# Autodesk Inventor assembly: chassis_assembly.ipt
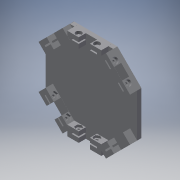
[picture p0: Inventor's stored thumbnail of the model, 180x180]
Saved by Autodesk Inventor 2018 (Build 220112000, 112)
## iProperties
Created: 2018-04-30
Part Number: chassis_assembly.ipt
Document SubType Name: Assembly
Designer: dvyen
Author: dvyen
## Documents named in this file (3)
- C:\Users\dvyen\source\repos\micromouse-2\drivetrain\chassis_assembly.ipt.iam
- C:\Users\dvyen\source\repos\micromouse-2\drivetrain\chassis.ipt
- C:\Users\dvyen\source\repos\micromouse-2\drivetrain\lidar_mount.ipt
## Components (7 placed, 2 different names)
1. chassis:1 — Mate:4, Mate:5, Mate:6, Mate:7, Mate:8, Mate:9, Mate:10, Mate:11, Mate:12, Mate:13, Mate:14, Mate:15, Mate:16, Mate:17, Mate:18, Mate:19, Mate:20, Mate:21
2. lidar_mount:3 — Mate:4, Mate:5, Mate:10
3. lidar_mount:6 — Mate:6, Mate:7, Mate:8, Mate:9
4. lidar_mount:7 — Mate:11, Mate:12
5. lidar_mount:8 — Mate:13, Mate:14, Mate:15
6. lidar_mount:9 — Mate:16, Mate:17, Mate:18
7. lidar_mount:10 — Mate:19, Mate:20, Mate:21
## Relationships (18: Mate 18)
- Mate:4: chassis:1 ↔ lidar_mount:3
- Mate:5: chassis:1 ↔ lidar_mount:3
- Mate:6: chassis:1 ↔ lidar_mount:6
- Mate:7: chassis:1 ↔ lidar_mount:6
- Mate:8: chassis:1 ↔ lidar_mount:6
- Mate:9: chassis:1 ↔ lidar_mount:6
- Mate:10: chassis:1 ↔ lidar_mount:3
- Mate:11: chassis:1 ↔ lidar_mount:7
- Mate:12: chassis:1 ↔ lidar_mount:7
- Mate:13: chassis:1 ↔ lidar_mount:8
- Mate:14: chassis:1 ↔ lidar_mount:8
- Mate:15: chassis:1 ↔ lidar_mount:8
- Mate:16: chassis:1 ↔ lidar_mount:9
- Mate:17: chassis:1 ↔ lidar_mount:9
- Mate:18: chassis:1 ↔ lidar_mount:9
- Mate:19: chassis:1 ↔ lidar_mount:10
- Mate:20: chassis:1 ↔ lidar_mount:10
- Mate:21: chassis:1 ↔ lidar_mount:10
